# Autodesk Inventor assembly: Assembly_2_servobox
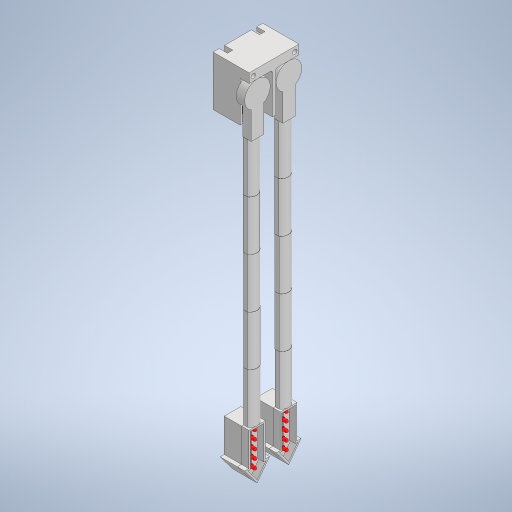
[picture p0: Inventor's stored thumbnail of the model, 512x512]
Saved by Autodesk Inventor 2023 (Build 270158000, 158)
## iProperties
Created: 2023-09-29
Part Number: Assembly_2_servobox
Document SubType Name: Assembly
Designer: zskus
Author: zskus
## Documents named in this file (7)
- C:\Users\zskus\Desktop\Folders\Personal Projects\Inventor\Project_1_Scooter\Assembly\Assembly_2_servobox.iam
- C:\Users\zskus\Desktop\Folders\Personal Projects\Inventor\Project_1_Scooter\Parts\Part_2_servobox.ipt
- C:\Users\zskus\Desktop\Folders\Personal Projects\Inventor\Project_1_Scooter\Parts\Part_3_hand.ipt
- C:\Users\zskus\Desktop\Folders\Personal Projects\Inventor\Project_1_Scooter\Parts\Part_3_hand_MIR.ipt
- C:\Users\zskus\Desktop\Folders\Personal Projects\Inventor\Project_1_Scooter\Parts\Servo Motor MG996R  With Attachments.iam
- C:\Users\zskus\Desktop\Folders\Personal Projects\Inventor\Project_1_Scooter\Parts\Servo Motor MG996R  With Attachments_MIR.iam
- C:\Users\zskus\Desktop\Folders\Personal Projects\Inventor\Project_1_Scooter\Assembly\Assembly6_arm.iam
## Components (7 placed, 6 different names)
1. Part_2_servobox:1 — Mate:4, Mate:39, Mate:40, Mate:41, Mate:45, Mate:46, Mate:47, Mate:49
2. Part_3_hand:1 — Mate:4, Mate:42, Mate:43, Mate:53, Mate:54, Mate:55
3. Part_3_hand_MIR:1 — Mate:44, Mate:48, Mate:49, Mate:50, Mate:51, Mate:52
4. Servo Motor MG996R  With Attachments:1 [sub-assembly] — Mate:39, Mate:40, Mate:41, Mate:42, Mate:43
5. Servo Motor MG996R  With Attachments_MIR:1 [sub-assembly] — Mate:44, Mate:45, Mate:46, Mate:47, Mate:48
6. Assembly6_arm:1 [sub-assembly] — Mate:50, Mate:51, Mate:52
7. Assembly6_arm:2 [sub-assembly] — Mate:53, Mate:54, Mate:55
## Relationships (18: Mate 18)
- Mate:4: Part_2_servobox:1 ↔ Part_3_hand:1
- Mate:39: Part_2_servobox:1 ↔ Servo Motor MG996R  With Attachments:1
- Mate:40: Part_2_servobox:1 ↔ Servo Motor MG996R  With Attachments:1
- Mate:41: Part_2_servobox:1 ↔ Servo Motor MG996R  With Attachments:1
- Mate:42: Part_3_hand:1 ↔ Servo Motor MG996R  With Attachments:1
- Mate:43: Part_3_hand:1 ↔ Servo Motor MG996R  With Attachments:1
- Mate:44: Part_3_hand_MIR:1 ↔ Servo Motor MG996R  With Attachments_MIR:1
- Mate:45: Part_2_servobox:1 ↔ Servo Motor MG996R  With Attachments_MIR:1
- Mate:46: Part_2_servobox:1 ↔ Servo Motor MG996R  With Attachments_MIR:1
- Mate:47: Part_2_servobox:1 ↔ Servo Motor MG996R  With Attachments_MIR:1
- Mate:48: Part_3_hand_MIR:1 ↔ Servo Motor MG996R  With Attachments_MIR:1
- Mate:49: Part_2_servobox:1 ↔ Part_3_hand_MIR:1
- Mate:50: Part_3_hand_MIR:1 ↔ Assembly6_arm:1
- Mate:51: Part_3_hand_MIR:1 ↔ Assembly6_arm:1
- Mate:52: Part_3_hand_MIR:1 ↔ Assembly6_arm:1
- Mate:53: Part_3_hand:1 ↔ Assembly6_arm:2
- Mate:54: Part_3_hand:1 ↔ Assembly6_arm:2
- Mate:55: Part_3_hand:1 ↔ Assembly6_arm:2
